# Autodesk Inventor assembly: PDRM50
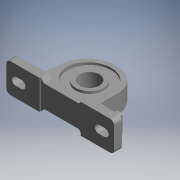
[picture p0: Inventor's stored thumbnail of the model, 180x180]
Saved by Autodesk Inventor 2017.3 (Build 213256000, 256)
## iProperties
Category: PARTsolutions
Company: MISUMI
Part Number: PDRM50
Catalog Web Link: www.cadenas.de
Description: PDRM-Ball Bearing Units - Pillow Casting Housing Type -
Vendor: MISUMI
Document SubType Name: Assembly
Designer: partserver
Manufacturer: MISUMI
Mass: 932.284 g
Surface Area: 1153.81 cm^2
Volume: 932.284 cm^3
Density: 1 g/cm^3
Title: PDRM50
Author: Cadenas PARTsolutions
Comments: Ball Bearing Units - Pillow Casting Housing Type -
PSOL_IDENT_0: {$CADENAS_DATA\23d-libs\misumi\metric\12_bearing_holders\pdrm_asmtab.prj},164 {VTYP=3D},{STYP=ASSTAB
PSOL_IDENT_1: },{NB=PDRM50},{LINA=PDRM50},{NN=PDRM},{DATE=18.09.2019 02:29:27},{GEOMDATE=03.09.2019 09:06:38},{VER
PSOL_IDENT_2: SION=},{LINEID=60},{WBVAR=},{WBNUMERIC=}  {NB=PDRM50},{LINA=PDRM50},{KT=DUMMY},{PN=PDRM50},{TYPE=PDR
PSOL_IDENT_3: M},{MTH=Alloy Cast Iron Class No.30},{MTB=52100 Bearing Steel},{MTRS=Silicon Rubber},{MTSS=4137 Allo
PSOL_IDENT_4: y Steel},{PRECISION=JIS B 1558, JIS B 1559},{OT=-15 ~+100},{D=50},{JIS=UCP310},{H=75},{L=275},{L1=21
PSOL_IDENT_5: 2},{A=75},{DD1=35},{DD=20},{TT=28},{H1=143},{B=61},{S=22},{CRR=61.5},{COR=38.2},{M1=M12x1.5},{M1ALG=
PSOL_IDENT_6: 12},{T=2790},{ALC=3075},{MASS=5680},{HR1=68},{HR2=111},{HR3=105.243},{HR4=70.5},{HH1=20},{HH2=23},{H
PSOL_IDENT_7: W2=89},{HW3=105},{HW4=143.0},{HA1=3.695},{HW5=56.5},{HW6=40},{R1=5},{R2=18},{R3=10},{LEN1=131.5},{LE
PSOL_IDENT_8: N2=18},{W=36},{BW=32},{GZ=9.0},{LS=12},{PPATH=pdrm/pdrm_asmtpl.prj}
NB: PDRM50
NN: PDRM
NT: Ball Bearing Units - Pillow Casting Housing Type -
NBSYN: $PN.
LINA: PDRM50
CATALOG: Misumi
PN: PDRM50
TYPE: PDRM
MTH: Alloy Cast Iron Class No.30
MTB: 52100 Bearing Steel
MTRS: Silicon Rubber
MTSS: 4137 Alloy Steel
PRECISION: JIS B 1558, JIS B 1559
OT: -15 ~+100
D: 50
JIS: UCP310
H: 75
L: 275
L1: 212
A: 75
DD1: 35
DD: 20
TT: 28
H1: 143
B: 61
S: 22
CRR: 61.5
COR: 38.2
M1: M12x1.5
T: 2790
ALC: 3075
MASS: 5680
PPATH: pdrm/pdrm_asmtpl.prj
SUPPLIER: MISUMI
ARTICLENO: PDRM50
BOMINFO: PDRM50
CREATOR: CADENAS GmbH
## Documents named in this file (3)
- e:\temp\worker_13\temp\exporttempdir_4908_354_kw0PR\format_0\PDRM50.iam
- e:\temp\worker_13\temp\exporttempdir_4908_354_kw0PR\format_0\PDRM50_b.ipt
- e:\temp\worker_13\temp\exporttempdir_4908_354_kw0PR\format_0\SET-SCREW12-12.ipt
## Components (3 placed, 2 different names)
1. PDRM50_b:1 — cp1_XY@1 <-> CP_XY@2, cp1_Z@1 <-> CP_Z@2, cp1_YZ@1 <-> CP_YZ@2, cp2_XY@1 <-> CP_XY@3, cp2_Z@1 <-> CP_Z@3, cp2_YZ@1 <-> CP_YZ@3
2. SET-SCREW12-12:1 — cp1_XY@1 <-> CP_XY@2, cp1_Z@1 <-> CP_Z@2, cp1_YZ@1 <-> CP_YZ@2
3. SET-SCREW12-12:2 — cp2_XY@1 <-> CP_XY@3, cp2_Z@1 <-> CP_Z@3, cp2_YZ@1 <-> CP_YZ@3
## Relationships (6: Mate 4, Angle 2)
- cp1_XY@1 <-> CP_XY@2 [Mate]: PDRM50_b:1 ↔ SET-SCREW12-12:1
- cp1_Z@1 <-> CP_Z@2 [Mate]: PDRM50_b:1 ↔ SET-SCREW12-12:1
- cp1_YZ@1 <-> CP_YZ@2 [Angle] (0 deg): PDRM50_b:1 ↔ SET-SCREW12-12:1
- cp2_XY@1 <-> CP_XY@3 [Mate]: PDRM50_b:1 ↔ SET-SCREW12-12:2
- cp2_Z@1 <-> CP_Z@3 [Mate]: PDRM50_b:1 ↔ SET-SCREW12-12:2
- cp2_YZ@1 <-> CP_YZ@3 [Angle] (0 deg): PDRM50_b:1 ↔ SET-SCREW12-12:2
